# Autodesk Inventor assembly: ASY PNS 1600 Filter column D1000
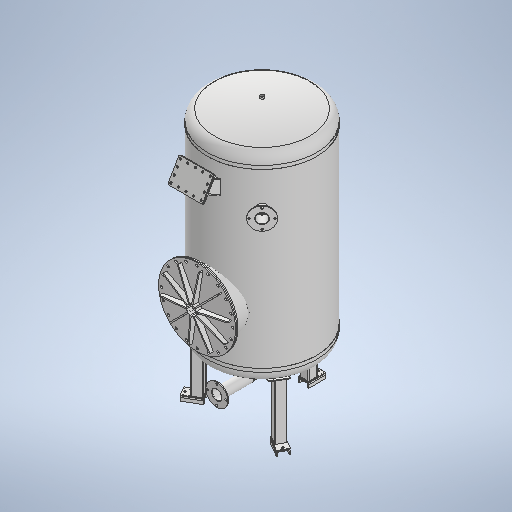
[picture p0: Inventor's stored thumbnail of the model, 512x512]
Saved by Autodesk Inventor 2025.4 (Build 294407000, 407)
## iProperties
allow_slope_adjustment: 0 ul
flow_configuration2: 1 ul
flow_direction: 2 ul
loss_method: 0 ul
radius: 45,500 mm
Created: 2025-02-13
Part Number: ASY PNS 1600 Filter column D1000
Document SubType Name: Assembly
Designer: pokla
Mass: 296006 g
Surface Area: 199460 cm^2
Volume: 66339.5 cm^3
Density: 4.46198 g/cm^3
radius: 16,750 mm
Author: pokla
Revision Number: 3
## Documents named in this file (23)
- C:\Users\admin\Documents\Inventor\SLM-Salemal\ASY SLM 1600 Filter column D940.iam
- C:\Users\admin\Documents\Inventor\SLM-Salemal\PNS-612 accses hatch flangeipt.ipt
- C:\Users\admin\Documents\Inventor\SLM-Salemal\PNS-611 accses hatch tube.ipt
- C:\Users\admin\Documents\Inventor\SLM-Salemal\PNS 1604 dished head D1000.ipt
- C:\Users\admin\Documents\Inventor\SLM-Salemal\Fitting G1.ipt
- C:\Users\admin\Documents\Inventor\SLM-Salemal\ASY PNS 1690 Filter legs D1000.iam
- C:\Users\admin\Documents\Inventor\SLM-Salemal\PNS 1633 charging blind flange.ipt
- C:\Users\admin\Documents\Inventor\SLM-Salemal\ASY PNS 1610 charging hatch.iam
- C:\Users\admin\Documents\Inventor\SLM-Salemal\cc\JIS B 2312 90 Deg Long Elbow Steel 80A x Sch 40.ipt
- C:\Users\admin\Documents\Inventor\SLM-Salemal\ASY PNS 1650 filter-distribution-system 1000.iam
- C:\Users\admin\Documents\Inventor\SLM-Salemal\PNS 1612 FDS tube 2.ipt
- C:\Users\admin\Documents\Inventor\SLM-Salemal\PNS 1606 charging flange round.ipt
- C:\Users\admin\Documents\Inventor\SLM-Salemal\PNS 1613 FDS tube 3.ipt
- C:\Users\admin\Documents\Inventor\SLM-Salemal\PNS 1614 FDS tube 4.ipt
- C:\Users\admin\Documents\Inventor\SLM-Salemal\PNS 1615 FDS tube 5.ipt
- C:\Users\admin\Documents\Inventor\SLM-Salemal\ASY PNS 179 top funnel 1200 50-90_1000x90.iam
- C:\Users\admin\Documents\Inventor\SLM-Salemal\pallet jack dummy.ipt
- C:\Users\admin\Documents\Inventor\SLM-Salemal\SLM 1431 FDS flange DN90.ipt
- C:\Users\admin\Documents\Inventor\SLM-Salemal\SLM 1432 FDS free flange DN90.ipt
- C:\Users\admin\Documents\Inventor\SLM-Salemal\SLM 1671 charging tube 1.ipt
- C:\Users\admin\Documents\Inventor\SLM-Salemal\SLM 1672 charging tube 2.ipt
- C:\Users\admin\Documents\Inventor\SLM-Salemal\PNS 1607 charging flange rect.ipt
- C:\Users\admin\Documents\Inventor\SLM-Salemal\PNS 9110 main Shell D 940.ipt
## Components (29 placed, 24 different names)
1. Fitting G1.ipt:1 — Rigid:15
2. PNS 1633 charging blind flange.ipt:2 — Rigid:67
3. ASY PNS 1650 filter-distribution-system 1000.iam:1 [sub-assembly] — Rotational:75
4. ASY PNS 179 top funnel 1200 50-90_1000x90:1 [sub-assembly] — Rotational:72
5. pallet jack dummy:1
6. PNS 1633 charging blind flange:5 — Rigid:77
7. PNS 1633 charging blind flange:6 — Rigid:78, Rotational:72
8. PNS 1604 dished head D1000.ipt:1 — Rigid:75, Rotational:77
9. Fitting G1.ipt:2 — Mate:4, Mate:5, Mate:6
10. JIS B 2312 90 Deg Long Elbow Steel 80A x Sch 40.ipt:1 — Rigid:68, Rigid:79, Mate:6
11. PNS 1613 FDS tube 3:1 — Rigid:67, Rigid:68, Flush:9
12. PNS 1614 FDS tube 4:1 — Rigid:79, Rigid:75, Rotational:71, Rotational:75
13. SLM 1431 FDS flange DN90:1 — Rigid:76
14. SLM 1432 FDS free flange DN90:1 — Rotational:71, Rigid:76
15. PNS-611 accses hatch tube.ipt:1 — Rotational:74, Rigid:85
16. PNS 1604 dished head D1000.ipt:2 — Rigid:15, Mate:3, Rotational:76
17. JIS B 2312 90 Deg Long Elbow Steel 80A x Sch 40.ipt:2 — Rigid:62, Rigid:73
18. PNS 1612 FDS tube 2:3 — Rigid:62, Rigid:78
19. PNS 1615 FDS tube 5:1 — Rigid:73, Rigid:77, Rigid:87
20. SLM 1672 charging tube 2:1 — Rigid:82, Rigid:84
21. SLM 1671 charging tube 1:1 — Rigid:84, Rigid:86
22. PNS 1606 charging flange round:1 — Rigid:82, Rigid:83
23. PNS 1607 charging flange rect:1 — Rigid:83
24. PNS-612 accses hatch flangeipt.ipt:1 — Rotational:73, Rotational:74
25. ASY PNS 1610 charging hatch.iam:1 [sub-assembly] — Rotational:73
26. PNS 9110 main Shell D 940:1 — Flush:7, Rigid:85, Flush:8, Rotational:76, Rotational:77, Rigid:86, Rigid:87
27. ASY PNS 1690 Filter legs D1000.iam:1 [sub-assembly] — Flush:2, Flush:10, Flush:11
28. ASY PNS 1690 Filter legs D1000:2 [sub-assembly]
29. ASY PNS 1690 Filter legs D1000:3 [sub-assembly]
## Component patterns: (3 elements, first: ASY PNS 1690 Filter legs D1000.iam:1)
## Relationships (33: WeldJoint 16, RevoluteJoint 7, Flush 6, Mate 4)
- Rigid:15 [WeldJoint]: Fitting G1.ipt:1 ↔ PNS 1604 dished head D1000.ipt:2
- Mate:3 (2350 mm): PNS 1604 dished head D1000.ipt:2
- Flush:2: ASY PNS 1690 Filter legs D1000.iam:1
- Rigid:62 [WeldJoint]: JIS B 2312 90 Deg Long Elbow Steel 80A x Sch 40.ipt:2 ↔ PNS 1612 FDS tube 2:3
- Rigid:67 [WeldJoint]: PNS 1633 charging blind flange.ipt:2 ↔ PNS 1613 FDS tube 3:1
- Rigid:68 [WeldJoint]: JIS B 2312 90 Deg Long Elbow Steel 80A x Sch 40.ipt:1 ↔ PNS 1613 FDS tube 3:1
- Rigid:79 [WeldJoint]: JIS B 2312 90 Deg Long Elbow Steel 80A x Sch 40.ipt:1 ↔ PNS 1614 FDS tube 4:1
- Rigid:73 [WeldJoint]: JIS B 2312 90 Deg Long Elbow Steel 80A x Sch 40.ipt:2 ↔ PNS 1615 FDS tube 5:1
- Rigid:75 [WeldJoint] (-50 mm): PNS 1604 dished head D1000.ipt:1 ↔ PNS 1614 FDS tube 4:1
- Rotational:71 [RevoluteJoint]: PNS 1614 FDS tube 4:1 ↔ SLM 1432 FDS free flange DN90:1
- Rigid:76 [WeldJoint]: SLM 1431 FDS flange DN90:1 ↔ SLM 1432 FDS free flange DN90:1
- Rigid:77 [WeldJoint]: PNS 1633 charging blind flange:5 ↔ PNS 1615 FDS tube 5:1
- Rigid:78 [WeldJoint]: PNS 1633 charging blind flange:6 ↔ PNS 1612 FDS tube 2:3
- Rotational:72 [RevoluteJoint]: ASY PNS 179 top funnel 1200 50-90_1000x90:1 ↔ PNS 1633 charging blind flange:6
- Rotational:73 [RevoluteJoint]: PNS-612 accses hatch flangeipt.ipt:1 ↔ ASY PNS 1610 charging hatch.iam:1
- Rotational:74 [RevoluteJoint]: PNS-611 accses hatch tube.ipt:1 ↔ PNS-612 accses hatch flangeipt.ipt:1
- Rotational:75 [RevoluteJoint]: ASY PNS 1650 filter-distribution-system 1000.iam:1 ↔ PNS 1614 FDS tube 4:1
- Rigid:82 [WeldJoint]: SLM 1672 charging tube 2:1 ↔ PNS 1606 charging flange round:1
- Rigid:83 [WeldJoint]: PNS 1606 charging flange round:1 ↔ PNS 1607 charging flange rect:1
- Rigid:84 [WeldJoint]: SLM 1672 charging tube 2:1 ↔ SLM 1671 charging tube 1:1
- Flush:10: ASY PNS 1690 Filter legs D1000.iam:1
- Flush:11: ASY PNS 1690 Filter legs D1000.iam:1
- Flush:7: PNS 9110 main Shell D 940:1
- Rigid:85 [WeldJoint]: PNS-611 accses hatch tube.ipt:1 ↔ PNS 9110 main Shell D 940:1
- Flush:8: PNS 9110 main Shell D 940:1
- Rotational:76 [RevoluteJoint]: PNS 1604 dished head D1000.ipt:2 ↔ PNS 9110 main Shell D 940:1
- Rotational:77 [RevoluteJoint]: PNS 1604 dished head D1000.ipt:1 ↔ PNS 9110 main Shell D 940:1
- Flush:9: PNS 1613 FDS tube 3:1
- Rigid:86 [WeldJoint]: SLM 1671 charging tube 1:1 ↔ PNS 9110 main Shell D 940:1
- Rigid:87 [WeldJoint] (100 mm): PNS 1615 FDS tube 5:1 ↔ PNS 9110 main Shell D 940:1
- Mate:4: Fitting G1.ipt:2
- Mate:5 (150 mm): Fitting G1.ipt:2
- Mate:6: Fitting G1.ipt:2 ↔ JIS B 2312 90 Deg Long Elbow Steel 80A x Sch 40.ipt:1
